# Autodesk Inventor assembly: RovoPitch
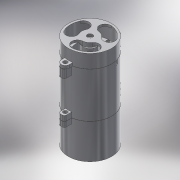
[picture p0: Inventor's stored thumbnail of the model, 180x180]
Saved by Autodesk Inventor 2018.2 (Build 222227000, 227)
## iProperties
Created: 2018-03-30
Part Number: RovoPitch
Document SubType Name: Assembly
Designer: Muchen He
Author: Muchen He
## Documents named in this file (5)
- C:\Users\Moochster\OneDrive\Documents\2018 UBC\ELEC 391\Controller\cad\release\PitchMotor\Rovo\RovoPitch.iam
- C:\Users\Moochster\OneDrive\Documents\2018 UBC\ELEC 391\Controller\cad\release\PitchMotor\Rovo\pitch_stator_front_attachment_flashlight_v2.ipt
- C:\Users\Moochster\OneDrive\Documents\2018 UBC\ELEC 391\Controller\cad\release\PitchMotor\Rovo\pitch_StatorShell_v5.ipt
- C:\Users\Moochster\OneDrive\Documents\2018 UBC\ELEC 391\Controller\cad\release\PitchMotor\Rovo\pitch_tube_commutator_attachment.ipt
- C:\Users\Moochster\OneDrive\Documents\2018 UBC\ELEC 391\Controller\cad\release\PitchMotor\Rovo\pitchThings.ipt
## Components (4 placed, 4 different names)
1. pitch_stator_front_attachment_flashlight_v2:1 — Mate:1, Mate:2, Mate:5, Flush:1, Mate:6, Mate:7, Mate:8
2. pitch_StatorShell_v5:1 — Mate:1, Mate:2, Mate:5
3. pitch_tube_commutator_attachment:1 — Flush:1
4. pitchThings:1 — Mate:6, Mate:7, Mate:8
## Relationships (7: Mate 6, Flush 1)
- Mate:1: pitch_stator_front_attachment_flashlight_v2:1 ↔ pitch_StatorShell_v5:1
- Mate:2: pitch_stator_front_attachment_flashlight_v2:1 ↔ pitch_StatorShell_v5:1
- Mate:5 (0.1 mm): pitch_stator_front_attachment_flashlight_v2:1 ↔ pitch_StatorShell_v5:1
- Flush:1 (-7 mm): pitch_stator_front_attachment_flashlight_v2:1 ↔ pitch_tube_commutator_attachment:1
- Mate:6 (0.1 mm): pitch_stator_front_attachment_flashlight_v2:1 ↔ pitchThings:1
- Mate:7: pitch_stator_front_attachment_flashlight_v2:1 ↔ pitchThings:1
- Mate:8: pitch_stator_front_attachment_flashlight_v2:1 ↔ pitchThings:1
